# Autodesk Inventor assembly: V-Slot Tnut Delrin Dual Wheel Eccentric Assembly
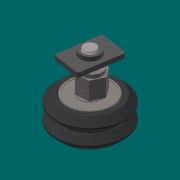
[picture p0: Inventor's stored thumbnail of the model, 180x180]
Saved by Autodesk Inventor 2016 (Build 200138000, 138)
## iProperties
Created: 2015-06-04
Part Number: V-Slot Tnut Delrin Dual Wheel Eccentric Assembly
Document SubType Name: Assembly
Designer: Sawaiz Syed
Author: Sawaiz Syed
## Documents named in this file (7)
- C:\Users\Sawaiz\Documents\data\projects\cncBlackBox\vWheel\V-Slot Tnut Delrin Dual Wheel Eccentric Assembly.iam
- C:\Users\Sawaiz\Documents\data\projects\cncBlackBox\hardware\delrinVWheel.ipt
- C:\Users\Sawaiz\Documents\data\projects\cncBlackBox\hardware\m5PrecisionWasher.ipt
- C:\Users\Sawaiz\Documents\data\projects\cncBlackBox\hardware\625BallBearing.ipt
- C:\Users\Sawaiz\Documents\data\projects\cncBlackBox\hardware\m5x25LowProfile.ipt
- C:\Users\Sawaiz\Documents\data\projects\cncBlackBox\hardware\eccentricSpacer.ipt
- C:\Users\Sawaiz\Documents\data\projects\cncBlackBox\hardware\m5TNut.ipt
## Components (7 placed, 6 different names)
1. delrinVWheel:1 — Mate:2, Flush:1, Mate:5, Mate:6, Mate:14, Flush:2, Mate:16
2. m5PrecisionWasher:1 — Flush:1, Flush:2, Mate:15
3. 625BallBearing:1 — Mate:5, Mate:11, Mate:13, Mate:14
4. 625BallBearing:2 — Mate:2, Mate:6, Mate:9
5. m5x25LowProfile:1 — Mate:9, Mate:12, Mate:13, Mate:15, Mate:16, Mate:17
6. eccentricSpacer:1 — Mate:11, Mate:12, Mate:18
7. m5TNut:1 — Mate:17, Mate:18
## Relationships (14: Mate 12, Flush 2)
- Mate:2: delrinVWheel:1 ↔ 625BallBearing:2
- Flush:1: delrinVWheel:1 ↔ m5PrecisionWasher:1
- Mate:5: delrinVWheel:1 ↔ 625BallBearing:1
- Mate:6: delrinVWheel:1 ↔ 625BallBearing:2
- Mate:9: 625BallBearing:2 ↔ m5x25LowProfile:1
- Mate:11: 625BallBearing:1 ↔ eccentricSpacer:1
- Mate:12: m5x25LowProfile:1 ↔ eccentricSpacer:1
- Mate:13: 625BallBearing:1 ↔ m5x25LowProfile:1
- Mate:14: delrinVWheel:1 ↔ 625BallBearing:1
- Flush:2: delrinVWheel:1 ↔ m5PrecisionWasher:1
- Mate:15: m5PrecisionWasher:1 ↔ m5x25LowProfile:1
- Mate:16: delrinVWheel:1 ↔ m5x25LowProfile:1
- Mate:17: m5x25LowProfile:1 ↔ m5TNut:1
- Mate:18 (4 mm): eccentricSpacer:1 ↔ m5TNut:1
